# Autodesk Inventor assembly: WindRotor
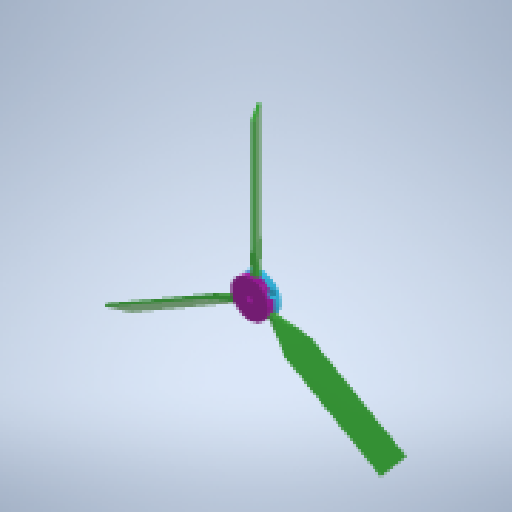
[picture p0: Inventor's stored thumbnail of the model, 512x512]
Saved by Autodesk Inventor 2024 (Build 280153000, 153)
## iProperties
Created: 2024-11-22
Part Number: WindRotor
Document SubType Name: Assembly
Designer: Maximilian Hock
Author: Maximilian Hock
## iProperties of the stored document MemberDocs/xU2w5zzgsEc4w2ofmJljfxw1lZa
Created: 2024-11-22
Part Number: WindRotor
Document SubType Name: Assembly
Designer: Maximilian Hock
Author: Maximilian Hock
## Documents named in this file (6)
- Y:\Dokumente\LearningKit\LearningKitWind\WindRotor.iam
- Y:\Dokumente\LearningKit\LearningKitWind\WindHub.ipt
- Y:\Dokumente\LearningKit\LearningKitWind\WindBladeFlat.ipt
- Z:\Dokumente\LearningKit\LearningKitWind\WindHub.ipt
- Z:\Dokumente\LearningKit\LearningKitWind\WindBlade.ipt
- Z:\Dokumente\LearningKit\LearningKitWind\WindBladeFlat.ipt
## Components (5 placed, 2 different names)
1. WindHub:1 — Passend:1, Passend:2, Winkel:1, Starr:2
2. WindHub:2 — Starr:2, Starr:3
3. WindBladeFlat:1 — Starr:3
4. WindBladeFlat:2
5. WindBladeFlat:3
## Component patterns: (3 elements, first: WindBladeFlat:1)
## Relationships (5: Mate 2, WeldJoint 2, Angle 1)
- Passend:1 [Mate]: WindHub:1
- Passend:2 [Mate]: WindHub:1
- Winkel:1 [Angle] (90 deg): WindHub:1
- Starr:2 [WeldJoint]: WindHub:1 ↔ WindHub:2
- Starr:3 [WeldJoint]: WindHub:2 ↔ WindBladeFlat:1
